# Autodesk Inventor assembly: Custom frame assembly
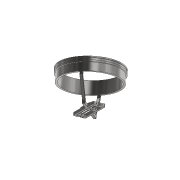
[picture p0: Inventor's stored thumbnail of the model, 180x180]
Saved by Autodesk Inventor 2020 (Build 240168000, 168)
## iProperties
Created: 2020-08-19
Part Number: Custom frame assembly
Document SubType Name: Assembly
Designer: ferrerx
Author: ferrerx
## Documents named in this file (6)
- C:\Users\ferrerx\Desktop\CALM Lab\Translational stages light sheet microscope\Inventor Design\Custom frame assembly.iam
- C:\Users\ferrerx\Desktop\CALM Lab\Translational stages light sheet microscope\Inventor Design\Custom_frame_1.ipt
- C:\Users\ferrerx\Desktop\CALM Lab\Translational stages light sheet microscope\Inventor Design\Moving platform.ipt
- C:\Users\ferrerx\Documents\Inventor\Content Center Files\R2020\en-US\AS 1474(1)\AS 1474 - M2(1).ipt
- C:\Users\ferrerx\Desktop\CALM Lab\Translational stages light sheet microscope\Inventor Design\ISOM2 x 50 mm.ipt
- C:\Users\ferrerx\Desktop\CALM Lab\Translational stages light sheet microscope\Inventor Design\M2 nut.ipt
## Components (7 placed, 4 different names)
1. Custom_frame_1:1 — Mate:7, Mate:21, Mate:22, Mate:23, Mate:24, Mate:25, Mate:26, Mate:27, Mate:28
2. Moving platform:1 — Mate:19, Mate:21, Mate:22
3. AS 1474 - Metric M2:1 — Mate:7, Mate:19
4. ISO 1580 M2 x 20:1 — Mate:23, Mate:24, Mate:29, Flush:1
5. ISO 1580 M2 x 20:2 — Mate:25, Mate:27
6. ISO 1580 M2 x 20:3 — Mate:26, Mate:28
7. AS 1474 - Metric M2:2 — Mate:29, Flush:1
## Relationships (12: Mate 11, Flush 1)
- Mate:7: Custom_frame_1:1 ↔ AS 1474 - Metric M2:1
- Mate:19: Moving platform:1 ↔ AS 1474 - Metric M2:1
- Mate:21: Custom_frame_1:1 ↔ Moving platform:1
- Mate:22: Custom_frame_1:1 ↔ Moving platform:1
- Mate:23: Custom_frame_1:1 ↔ ISO 1580 M2 x 20:1
- Mate:24: Custom_frame_1:1 ↔ ISO 1580 M2 x 20:1
- Mate:25: Custom_frame_1:1 ↔ ISO 1580 M2 x 20:2
- Mate:26: Custom_frame_1:1 ↔ ISO 1580 M2 x 20:3
- Mate:27: Custom_frame_1:1 ↔ ISO 1580 M2 x 20:2
- Mate:28: Custom_frame_1:1 ↔ ISO 1580 M2 x 20:3
- Mate:29: ISO 1580 M2 x 20:1 ↔ AS 1474 - Metric M2:2
- Flush:1: ISO 1580 M2 x 20:1 ↔ AS 1474 - Metric M2:2
